# Autodesk Inventor assembly: Arduino UNO R3 screw Shield v2 Left
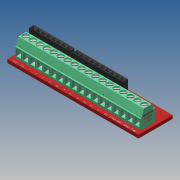
[picture p0: Inventor's stored thumbnail of the model, 180x180]
Saved by Autodesk Inventor 2017 SP1 (Build 210196100, 196)
## iProperties
Created: 2022-11-07
Part Number: Arduino UNO R3 screw Shield v2 Left
Document SubType Name: Assembly
Designer: Antonio
Author: Antonio
## Documents named in this file (7)
- C:\Users\Antonio\Documents\Inventor\Secador v2\Arduino UNO R3 screw shield v2\Arduino UNO R3 screw Shield v2 Left.iam
- C:\Users\Antonio\Documents\Inventor\Secador v2\DG381-3.5-06P-14-00AH.ipt
- C:\Users\Antonio\Documents\Inventor\Secador v2\HEMBRA 8 PINESB.ipt
- C:\Users\Antonio\Documents\Inventor\Secador v2\hembra 10 pines.ipt
- C:\Users\Antonio\Documents\Inventor\Secador v2\Pin Header 1x8 TH Pitch 2.54mm.ipt
- C:\Users\Antonio\Documents\Inventor\Secador v2\Pin Header 1x10 TH Pitch 2.54mm.ipt
- C:\Users\Antonio\Documents\Inventor\Secador v2\Arduino UNO R3 screw shield v2\Arduino UNO R3 screw shield v2 board Left.ipt
## Components (8 placed, 6 different names)
1. DG381-3.5-06P-14-00AH:1 — Coincidencia:3, Coincidencia:11
2. DG381-3.5-06P-14-00AH:2 — Coincidencia:3, Coincidencia:5, Nivelación:4, Nivelación:13
3. DG381-3.5-06P-14-00AH:3 — Coincidencia:5, Nivelación:4, Nivelación:12
4. HEMBRA 8 PINESB:1 — Coincidencia:7, Nivelación:7, Nivelación:8
5. hembra 10 pines:1 — Coincidencia:7, Nivelación:7, Nivelación:8
6. Pin Header 1x8 TH Pitch 2.54mm:1 — Coincidencia:10, Nivelación:11
7. Pin Header 1x10 TH Pitch 2.54mm:1 — Coincidencia:10, Nivelación:11
8. Arduino UNO R3 screw shield v2 board Left:1 — Coincidencia:11, Nivelación:12, Nivelación:13
## Relationships (11: Flush 6, Mate 5)
- Coincidencia:3 [Mate]: DG381-3.5-06P-14-00AH:1 ↔ DG381-3.5-06P-14-00AH:2
- Coincidencia:5 [Mate]: DG381-3.5-06P-14-00AH:2 ↔ DG381-3.5-06P-14-00AH:3
- Nivelación:4 [Flush]: DG381-3.5-06P-14-00AH:2 ↔ DG381-3.5-06P-14-00AH:3
- Coincidencia:7 [Mate] (1.55 mm): HEMBRA 8 PINESB:1 ↔ hembra 10 pines:1
- Nivelación:7 [Flush]: HEMBRA 8 PINESB:1 ↔ hembra 10 pines:1
- Nivelación:8 [Flush]: HEMBRA 8 PINESB:1 ↔ hembra 10 pines:1
- Coincidencia:10 [Mate] (1.55 mm): Pin Header 1x8 TH Pitch 2.54mm:1 ↔ Pin Header 1x10 TH Pitch 2.54mm:1
- Nivelación:11 [Flush]: Pin Header 1x8 TH Pitch 2.54mm:1 ↔ Pin Header 1x10 TH Pitch 2.54mm:1
- Coincidencia:11 [Mate]: DG381-3.5-06P-14-00AH:1 ↔ Arduino UNO R3 screw shield v2 board Left:1
- Nivelación:12 [Flush] (-1.48 mm): DG381-3.5-06P-14-00AH:3 ↔ Arduino UNO R3 screw shield v2 board Left:1
- Nivelación:13 [Flush] (-2.5 mm): DG381-3.5-06P-14-00AH:2 ↔ Arduino UNO R3 screw shield v2 board Left:1
